# Autodesk Inventor assembly: Camera
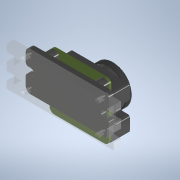
[picture p0: Inventor's stored thumbnail of the model, 180x180]
Saved by Autodesk Inventor 2020 (Build 240168000, 168)
## iProperties
Created: 2019-08-05
Part Number: Camera
Document SubType Name: Assembly
Designer: n10208577
Author: n10208577
## Documents named in this file (6)
- C:\Users\n10208577\Desktop\DRC\DRC2020-Hardware\Design\Camera.iam
- C:\Users\n10208577\Desktop\DRC\DRC2020-Hardware\Design\lense.ipt
- C:\Users\n10208577\Desktop\DRC\DRC2020-Hardware\Design\rpiCam.ipt
- C:\Users\n10208577\Desktop\DRC\DRC2020-Hardware\Design\rpiCamM12Mount.ipt
- C:\Users\n10208577\Desktop\DRC\DRC2020-Hardware\Design\rpiCamMount.ipt
- C:\Users\n10208577\Desktop\DRC\DRC2020-Hardware\Design\camMountBacking.ipt
## Components (5 placed, 5 different names)
1. lense:1 — Insert:3
2. rpiCam:1 — Insert:1, Insert:2, Insert:4, Insert:5
3. rpiCamM12Mount:1 — Insert:1, Insert:2, Insert:3
4. rpiCamMount:1 — Insert:4, Insert:5, Insert:6, Insert:7
5. camMountBacking:1 — Insert:6, Insert:7
## Relationships (7: Insert 7)
- Insert:1: rpiCam:1 ↔ rpiCamM12Mount:1
- Insert:2: rpiCam:1 ↔ rpiCamM12Mount:1
- Insert:3: lense:1 ↔ rpiCamM12Mount:1
- Insert:4: rpiCam:1 ↔ rpiCamMount:1
- Insert:5: rpiCam:1 ↔ rpiCamMount:1
- Insert:6: rpiCamMount:1 ↔ camMountBacking:1
- Insert:7: rpiCamMount:1 ↔ camMountBacking:1
